# Autodesk Inventor assembly: GFRP_T2_16
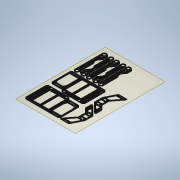
[picture p0: Inventor's stored thumbnail of the model, 180x180]
Saved by Autodesk Inventor 2020 (Build 240168000, 168)
## iProperties
Created: 2021-08-27
Part Number: GFRP_T2_16
Document SubType Name: Assembly
Designer: Masato
Author: Masato
## Documents named in this file (5)
- C:\Inventor\SUSTAINA-OP\Cam\GFRP_T2_16.iam
- C:\Inventor\SUSTAINA-OP\Cam\DisposableBoard.ipt
- C:\Inventor\SUSTAINA-OP\UpperBody\Trunk\Trunk_upper_side_frame.ipt
- C:\Inventor\SUSTAINA-OP\UpperBody\Head\Head_side_frame.ipt
- C:\Inventor\SUSTAINA-OP\LowerBody\Link\BackLink_frame.ipt
## Components (10 placed, 4 different names)
1. DisposableBoard:1 — メイト:2, メイト:1, フラッシュ:1, フラッシュ:2, メイト:4, メイト:5, フラッシュ:3, フラッシュ:4, メイト:7, メイト:9, メイト:12, メイト:13, フラッシュ:8, フラッシュ:9, メイト:15
2. Trunk_upper_side_frame:1 — メイト:4, フラッシュ:3, フラッシュ:4, メイト:6, フラッシュ:5, フラッシュ:6, メイト:8
3. Trunk_upper_side_frame:2 — メイト:5, メイト:6, フラッシュ:5, 正接:1, 正接:2, 正接:3
4. Head_side_frame:1 — メイト:7, フラッシュ:6, メイト:8, メイト:10
5. Head_side_frame:2 — メイト:9, メイト:10, フラッシュ:8
6. BackLink_frame:5 — メイト:15, メイト:16, 正接:3
7. BackLink_frame:1 — メイト:12, メイト:14, 正接:1, フラッシュ:9
8. BackLink_frame:2 — メイト:13, メイト:14, 正接:2
9. BackLink_frame:3
10. BackLink_frame:4 — メイト:16
## Component patterns: (2 elements, first: BackLink_frame:1 + BackLink_frame:2)
## Relationships (25: Mate 14, Flush 8, Tangent 3)
- メイト:2 [Mate]: DisposableBoard:1
- メイト:1 [Mate]: DisposableBoard:1
- フラッシュ:1 [Flush]: DisposableBoard:1
- フラッシュ:2 [Flush]: DisposableBoard:1
- メイト:4 [Mate]: DisposableBoard:1 ↔ Trunk_upper_side_frame:1
- メイト:5 [Mate]: DisposableBoard:1 ↔ Trunk_upper_side_frame:2
- フラッシュ:3 [Flush] (-2.5 mm): DisposableBoard:1 ↔ Trunk_upper_side_frame:1
- フラッシュ:4 [Flush] (3.5 mm): DisposableBoard:1 ↔ Trunk_upper_side_frame:1
- メイト:6 [Mate] (2.5 mm): Trunk_upper_side_frame:1 ↔ Trunk_upper_side_frame:2
- フラッシュ:5 [Flush]: Trunk_upper_side_frame:1 ↔ Trunk_upper_side_frame:2
- メイト:7 [Mate]: DisposableBoard:1 ↔ Head_side_frame:1
- フラッシュ:6 [Flush]: Trunk_upper_side_frame:1 ↔ Head_side_frame:1
- メイト:8 [Mate] (2.5 mm): Trunk_upper_side_frame:1 ↔ Head_side_frame:1
- メイト:9 [Mate]: DisposableBoard:1 ↔ Head_side_frame:2
- メイト:10 [Mate] (2.5 mm): Head_side_frame:1 ↔ Head_side_frame:2
- メイト:12 [Mate]: DisposableBoard:1 ↔ BackLink_frame:1
- メイト:13 [Mate]: DisposableBoard:1 ↔ BackLink_frame:2
- メイト:14 [Mate] (2.5 mm): BackLink_frame:1 ↔ BackLink_frame:2
- 正接:1 [Tangent] (2.5 mm): Trunk_upper_side_frame:2 ↔ BackLink_frame:1
- 正接:2 [Tangent] (2.5 mm): Trunk_upper_side_frame:2 ↔ BackLink_frame:2
- フラッシュ:8 [Flush] (2.5 mm): DisposableBoard:1 ↔ Head_side_frame:2
- フラッシュ:9 [Flush] (5 mm): DisposableBoard:1 ↔ BackLink_frame:1
- メイト:15 [Mate]: DisposableBoard:1 ↔ BackLink_frame:5
- メイト:16 [Mate] (2.5 mm): BackLink_frame:5 ↔ BackLink_frame:4
- 正接:3 [Tangent] (2.5 mm): Trunk_upper_side_frame:2 ↔ BackLink_frame:5
